# Autodesk Inventor assembly: 1678-16-A-0800
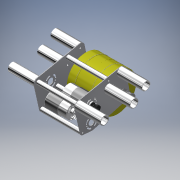
[picture p0: Inventor's stored thumbnail of the model, 180x180]
Saved by Autodesk Inventor 2019 (Build 230136000, 136)
## iProperties
Created: 2018-10-31
Part Number: 1678-16-A-0800
Document SubType Name: Assembly
Designer: woodk
Author: woodk
Revision Number: ANY
## Documents named in this file (14)
- F:\adrian-frc-team-1678-2016-1.snapshot.20\1678-16-A-0800.iam
- F:\adrian-frc-team-1678-2016-1.snapshot.20\1678-16-P-0801 - Copy.ipt
- F:\adrian-frc-team-1678-2016-1.snapshot.20\1678-16-P-0803 - Copy.ipt
- F:\adrian-frc-team-1678-2016-1.snapshot.20\bearing_fr8_.5hex.ipt
- F:\adrian-frc-team-1678-2016-1.snapshot.20\motor_775pro.ipt
- F:\adrian-frc-team-1678-2016-1.snapshot.20\pulley_12t_gt2_3mmp_9mmw_775propinion.ipt
- F:\adrian-frc-team-1678-2016-1.snapshot.20\pulley_30t_gt2_3mmp_9mmw_dblflange.ipt
- F:\adrian-frc-team-1678-2016-1.snapshot.20\Mirrorpulley_30t_gt2_3mmp_9mmw_dblflange.ipt
- F:\adrian-frc-team-1678-2016-1.snapshot.20\1678-16-P-0806.ipt
- F:\adrian-frc-team-1678-2016-1.snapshot.20\EE_Encoder_US Digital.ipt
- F:\adrian-frc-team-1678-2016-1.snapshot.20\1678-16-P-0809.ipt
- F:\adrian-frc-team-1678-2016-1.snapshot.20\1678-16-P-0812.ipt
- F:\adrian-frc-team-1678-2016-1.snapshot.20\1678-16-P-0811.ipt
- F:\adrian-frc-team-1678-2016-1.snapshot.20\1678-16-P-0815.ipt
## Components (26 placed, 26 different names)
1. 1678-16-P-0801 - Copy_179 — Insert:4, Insert:5, Insert:6, Insert:7, Insert:10, Insert:11, Insert:12, Insert:15, Insert:17, Mate:11
2. 1678-16-P-0803 - Copy_180 — Mate:4, Mate:5, Mate:7
3. bearing_fr8_.5hex_181 — Insert:17, Mate:4, Mate:5, Mate:12
4. 1678-16-P-0801 - Copy_182 — Insert:1, Insert:2, Insert:3, Insert:8, Insert:9, Insert:13, Insert:14, Insert:16, Insert:18
5. bearing_fr8_.5hex_183 — Insert:18, Mate:3, Mate:6
6. motor_775pro_184 — Flush:1, Mate:2, Insert:15
7. pulley_12t_gt2_3mmp_9mmw_775propinion_185 — Flush:1, Mate:2
8. pulley_30t_gt2_3mmp_9mmw_dblflange_186 — Mate:10, Flush:4
9. Mirrorpulley_30t_gt2_3mmp_9mmw_dblflange_187 — Mate:9, Flush:3, Mate:12
10. 1678-16-P-0806_188 — Mate:9, Flush:3, Mate:10, Flush:4, Insert:19, Mate:11
11. EE_Encoder_US Digital_189 — Insert:19
12. 1678-16-P-0809_190 — Insert:12, Insert:14
13. 1678-16-P-0809_191 — Insert:7, Insert:8
14. 1678-16-P-0809_192 — Insert:9, Insert:10
15. motor_775pro_193 — Flush:2, Mate:1, Insert:16
16. pulley_12t_gt2_3mmp_9mmw_775propinion_194 — Flush:2, Mate:1
17. 1678-16-P-0809_195 — Insert:11, Insert:13
18. 1678-16-P-0812_196 — Insert:6
19. 1678-16-P-0811_197 — Insert:4
20. 1678-16-P-0811_198 — Insert:5
21. 1678-16-P-0811_199 — Insert:1
22. 1678-16-P-0811_200 — Insert:2
23. 1678-16-P-0812_201 — Insert:3
24. 1678-16-P-0803 - Copy_202 — Mate:3, Mate:6, Mate:8
25. 1678-16-P-0815_203 — Mate:8
26. 1678-16-P-0815_204 — Mate:7
## Relationships (35: Insert 19, Mate 12, Flush 4)
- Insert:1: 1678-16-P-0801 - Copy_182 ↔ 1678-16-P-0811_199
- Insert:2: 1678-16-P-0801 - Copy_182 ↔ 1678-16-P-0811_200
- Insert:3: 1678-16-P-0801 - Copy_182 ↔ 1678-16-P-0812_201
- Insert:4: 1678-16-P-0801 - Copy_179 ↔ 1678-16-P-0811_197
- Insert:5: 1678-16-P-0801 - Copy_179 ↔ 1678-16-P-0811_198
- Insert:6: 1678-16-P-0801 - Copy_179 ↔ 1678-16-P-0812_196
- Insert:7: 1678-16-P-0801 - Copy_179 ↔ 1678-16-P-0809_191
- Insert:8: 1678-16-P-0801 - Copy_182 ↔ 1678-16-P-0809_191
- Insert:9: 1678-16-P-0801 - Copy_182 ↔ 1678-16-P-0809_192
- Insert:10: 1678-16-P-0801 - Copy_179 ↔ 1678-16-P-0809_192
- Insert:11: 1678-16-P-0801 - Copy_179 ↔ 1678-16-P-0809_195
- Insert:12: 1678-16-P-0801 - Copy_179 ↔ 1678-16-P-0809_190
- Insert:13: 1678-16-P-0801 - Copy_182 ↔ 1678-16-P-0809_195
- Insert:14: 1678-16-P-0801 - Copy_182 ↔ 1678-16-P-0809_190
- Flush:1 (-9.7028 mm): motor_775pro_184 ↔ pulley_12t_gt2_3mmp_9mmw_775propinion_185
- Flush:2 (-9.7028 mm): motor_775pro_193 ↔ pulley_12t_gt2_3mmp_9mmw_775propinion_194
- Mate:1: motor_775pro_193 ↔ pulley_12t_gt2_3mmp_9mmw_775propinion_194
- Mate:2: motor_775pro_184 ↔ pulley_12t_gt2_3mmp_9mmw_775propinion_185
- Insert:15: 1678-16-P-0801 - Copy_179 ↔ motor_775pro_184
- Insert:16: 1678-16-P-0801 - Copy_182 ↔ motor_775pro_193
- Insert:17: 1678-16-P-0801 - Copy_179 ↔ bearing_fr8_.5hex_181
- Insert:18: 1678-16-P-0801 - Copy_182 ↔ bearing_fr8_.5hex_183
- Mate:3 (8.636 mm): bearing_fr8_.5hex_183 ↔ 1678-16-P-0803 - Copy_202
- Mate:4 (8.636 mm): 1678-16-P-0803 - Copy_180 ↔ bearing_fr8_.5hex_181
- Mate:5: 1678-16-P-0803 - Copy_180 ↔ bearing_fr8_.5hex_181
- Mate:6: bearing_fr8_.5hex_183 ↔ 1678-16-P-0803 - Copy_202
- Mate:7: 1678-16-P-0803 - Copy_180 ↔ 1678-16-P-0815_204
- Mate:8: 1678-16-P-0803 - Copy_202 ↔ 1678-16-P-0815_203
- Mate:9: Mirrorpulley_30t_gt2_3mmp_9mmw_dblflange_187 ↔ 1678-16-P-0806_188
- Flush:3: Mirrorpulley_30t_gt2_3mmp_9mmw_dblflange_187 ↔ 1678-16-P-0806_188
- Mate:10: pulley_30t_gt2_3mmp_9mmw_dblflange_186 ↔ 1678-16-P-0806_188
- Flush:4: pulley_30t_gt2_3mmp_9mmw_dblflange_186 ↔ 1678-16-P-0806_188
- Insert:19: 1678-16-P-0806_188 ↔ EE_Encoder_US Digital_189
- Mate:11: 1678-16-P-0801 - Copy_179 ↔ 1678-16-P-0806_188
- Mate:12 (1.5875 mm): bearing_fr8_.5hex_181 ↔ Mirrorpulley_30t_gt2_3mmp_9mmw_dblflange_187
